# Autodesk Inventor assembly: 110033226_iam_11_農田
(part 2 of 2)
- 貼合:17 [Mate]: 110033226_ipt_44_農田基地:3 ↔ 110033226_ipt_21_柵欄:16
- 貼合:18 [Mate]: 110033226_ipt_44_農田基地:3 ↔ 110033226_ipt_21_柵欄:14
- 貼合:19 [Mate]: 110033226_ipt_44_農田基地:3 ↔ 110033226_ipt_21_柵欄:14
- 貼合:20 [Mate]: 110033226_ipt_04_小河:3 ↔ 110033226_ipt_21_柵欄:14
- 貼合:21 [Mate]: 110033226_ipt_44_農田基地:3 ↔ 110033226_ipt_21_柵欄:15
- 貼合:22 [Mate]: 110033226_ipt_44_農田基地:3 ↔ 110033226_ipt_21_柵欄:15
- 貼合:23 [Mate]: 110033226_ipt_04_小河:15 ↔ 110033226_ipt_21_柵欄:15
- 貼合:24 [Mate]: 110033226_ipt_44_農田基地:3 ↔ 110033226_ipt_07_磚塊樺木(2x1):1
- 貼合:25 [Mate]: 110033226_ipt_44_農田基地:3 ↔ 110033226_ipt_07_磚塊樺木(2x1):1
- 貼合:26 [Mate]: 110033226_ipt_44_農田基地:3 ↔ 110033226_ipt_07_磚塊樺木(2x1):1
- 貼合:27 [Mate]: 110033226_ipt_44_農田基地:3 ↔ 110033226_ipt_07_磚塊樺木(2x1):3
- 貼合:28 [Mate]: 110033226_ipt_44_農田基地:3 ↔ 110033226_ipt_07_磚塊樺木(2x1):3
- 貼合:29 [Mate]: 110033226_ipt_44_農田基地:3 ↔ 110033226_ipt_07_磚塊樺木(2x1):3
- 貼合:30 [Mate]: 110033226_ipt_44_農田基地:3 ↔ 110033226_ipt_07_磚塊樺木(2x1):5
- 貼合:31 [Mate]: 110033226_ipt_44_農田基地:3 ↔ 110033226_ipt_07_磚塊樺木(2x1):5
- 貼合:32 [Mate]: 110033226_ipt_44_農田基地:3 ↔ 110033226_ipt_07_磚塊樺木(2x1):5
- 貼合:33 [Mate]: 110033226_ipt_44_農田基地:3 ↔ 110033226_ipt_07_磚塊樺木(2x1):2
- 貼合:34 [Mate]: 110033226_ipt_44_農田基地:3 ↔ 110033226_ipt_07_磚塊樺木(2x1):2
- 貼合:35 [Mate]: 110033226_ipt_44_農田基地:3 ↔ 110033226_ipt_07_磚塊樺木(2x1):2
- 貼合:36 [Mate]: 110033226_ipt_44_農田基地:3 ↔ 110033226_ipt_07_磚塊樺木(2x1):4
- 貼合:37 [Mate]: 110033226_ipt_44_農田基地:3 ↔ 110033226_ipt_07_磚塊樺木(2x1):4
- 貼合:38 [Mate]: 110033226_ipt_44_農田基地:3 ↔ 110033226_ipt_07_磚塊樺木(2x1):4
- 貼合:39 [Mate]: 110033226_ipt_44_農田基地:3 ↔ 110033226_ipt_13_草地二:1
- 貼合:40 [Mate]: 110033226_ipt_44_農田基地:3 ↔ 110033226_ipt_13_草地二:1
- 貼合:41 [Mate]: 110033226_ipt_44_農田基地:3 ↔ 110033226_ipt_13_草地二:1
- 貼合:42 [Mate]: 110033226_ipt_44_農田基地:3 ↔ 110033226_ipt_13_草地二:12
- 貼合:43 [Mate]: 110033226_ipt_44_農田基地:3 ↔ 110033226_ipt_13_草地二:12
- 貼合:44 [Mate]: 110033226_ipt_44_農田基地:3 ↔ 110033226_ipt_13_草地二:12
- 貼合:45 [Mate]: 110033226_ipt_44_農田基地:3 ↔ 110033226_ipt_13_草地二:11
- 貼合:46 [Mate]: 110033226_ipt_44_農田基地:3 ↔ 110033226_ipt_13_草地二:11
- 貼合:47 [Mate]: 110033226_ipt_44_農田基地:3 ↔ 110033226_ipt_13_草地二:11
- 貼合:48 [Mate]: 110033226_ipt_44_農田基地:3 ↔ 110033226_ipt_07_磚塊樺木(2x1):38
- 貼合:49 [Mate]: 110033226_ipt_44_農田基地:3 ↔ 110033226_ipt_07_磚塊樺木(2x1):38
- 貼合:50 [Mate]: 110033226_ipt_44_農田基地:3 ↔ 110033226_ipt_06_磚塊樺木(1x1):3
- 貼合:51 [Mate]: 110033226_ipt_07_磚塊樺木(2x1):38 ↔ 110033226_ipt_06_磚塊樺木(1x1):3
- 貼合:52 [Mate]: 110033226_ipt_07_磚塊樺木(2x1):38 ↔ 110033226_ipt_06_磚塊樺木(1x1):3
- 貼合:53 [Mate]: 110033226_ipt_06_磚塊樺木(1x1):11 ↔ 110033226_ipt_07_磚塊樺木(2x1):36
- 貼合:54 [Mate]: 110033226_ipt_06_磚塊樺木(1x1):11 ↔ 110033226_ipt_07_磚塊樺木(2x1):36
- 貼合:55 [Mate]: 110033226_ipt_07_磚塊樺木(2x1):46 ↔ 110033226_ipt_07_磚塊樺木(2x1):36
- 貼合:56 [Mate]: 110033226_ipt_07_磚塊樺木(2x1):46 ↔ 110033226_ipt_06_磚塊樺木(1x1):1
- 貼合:57 [Mate]: 110033226_ipt_07_磚塊樺木(2x1):36 ↔ 110033226_ipt_06_磚塊樺木(1x1):1
- 貼合:58 [Mate]: 110033226_ipt_07_磚塊樺木(2x1):36 ↔ 110033226_ipt_06_磚塊樺木(1x1):1
- 貼合:59 [Mate]: 110033226_ipt_06_磚塊樺木(1x1):10 ↔ 110033226_ipt_07_磚塊樺木(2x1):37
- 貼合:60 [Mate]: 110033226_ipt_06_磚塊樺木(1x1):9 ↔ 110033226_ipt_07_磚塊樺木(2x1):37
- 貼合:61 [Mate]: 110033226_ipt_06_磚塊樺木(1x1):10 ↔ 110033226_ipt_07_磚塊樺木(2x1):37
- 貼合:62 [Mate]: 110033226_ipt_06_磚塊樺木(1x1):8 ↔ 110033226_ipt_06_磚塊樺木(1x1):2
- 貼合:63 [Mate]: 110033226_ipt_06_磚塊樺木(1x1):8 ↔ 110033226_ipt_06_磚塊樺木(1x1):2
- 貼合:64 [Mate]: 110033226_ipt_06_磚塊樺木(1x1):8 ↔ 110033226_ipt_06_磚塊樺木(1x1):2
- 貼合:65 [Mate]: 110033226_ipt_06_磚塊樺木(1x1):96 ↔ 110033226_ipt_07_磚塊樺木(2x1):144
- 貼合:66 [Mate]: 110033226_ipt_06_磚塊樺木(1x1):96 ↔ 110033226_ipt_07_磚塊樺木(2x1):144
- 貼合:67 [Mate]: 110033226_ipt_07_磚塊樺木(2x1):143 ↔ 110033226_ipt_07_磚塊樺木(2x1):144
- 貼合:68 [Mate]: 110033226_ipt_07_磚塊樺木(2x1):65 ↔ 110033226_ipt_07_磚塊樺木(2x1):184
- 貼合:69 [Mate]: 110033226_ipt_07_磚塊樺木(2x1):56 ↔ 110033226_ipt_07_磚塊樺木(2x1):184
- 貼合:70 [Mate]: 110033226_ipt_07_磚塊樺木(2x1):65 ↔ 110033226_ipt_07_磚塊樺木(2x1):184
- 貼合:71 [Mate]: 110033226_ipt_07_磚塊樺木(2x1):56 ↔ 110033226_ipt_06_磚塊樺木(1x1):133
- 貼合:72 [Mate]: 110033226_ipt_07_磚塊樺木(2x1):56 ↔ 110033226_ipt_06_磚塊樺木(1x1):133
- 貼合:73 [Mate]: 110033226_ipt_07_磚塊樺木(2x1):56 ↔ 110033226_ipt_06_磚塊樺木(1x1):133
- 貼合:74 [Mate]: 110033226_ipt_07_磚塊樺木(2x1):84 ↔ 110033226_ipt_12_平滑面(2x1):1
- 貼合:75 [Mate]: 110033226_ipt_07_磚塊樺木(2x1):84 ↔ 110033226_ipt_12_平滑面(2x1):1
- 貼合:76 [Mate]: 110033226_ipt_07_磚塊樺木(2x1):84 ↔ 110033226_ipt_12_平滑面(2x1):1
- 貼合:77 [Mate]: 110033226_ipt_07_磚塊樺木(2x1):38 ↔ 110033226_ipt_08_平滑面(3x1):1
- 貼合:78 [Mate]: 110033226_ipt_07_磚塊樺木(2x1):47 ↔ 110033226_ipt_08_平滑面(3x1):1
- 貼合:79 [Mate]: 110033226_ipt_08_平滑面(3x1):1 ↔ 110033226_ipt_06_磚塊樺木(1x1):97
- 貼合:80 [Mate]: 110033226_ipt_07_磚塊樺木(2x1):47 ↔ 110033226_ipt_08_平滑面(3x1):9
- 貼合:81 [Mate]: 110033226_ipt_07_磚塊樺木(2x1):47 ↔ 110033226_ipt_08_平滑面(3x1):9
- 貼合:82 [Mate]: 110033226_ipt_06_磚塊樺木(1x1):26 ↔ 110033226_ipt_08_平滑面(3x1):11
- 貼合:83 [Mate]: 110033226_ipt_06_磚塊樺木(1x1):50 ↔ 110033226_ipt_08_平滑面(3x1):11
- 貼合:84 [Mate]: 110033226_ipt_06_磚塊樺木(1x1):50 ↔ 110033226_ipt_08_平滑面(3x1):11
- 貼合:85 [Mate]: 110033226_ipt_07_磚塊樺木(2x1):54 ↔ 110033226_ipt_07_磚塊樺木(2x1):208
- 貼合:86 [Mate]: 110033226_ipt_07_磚塊樺木(2x1):53 ↔ 110033226_ipt_07_磚塊樺木(2x1):208
- 貼合:87 [Mate]: 110033226_ipt_07_磚塊樺木(2x1):54 ↔ 110033226_ipt_07_磚塊樺木(2x1):208
- 貼合:88 [Mate]: 110033226_ipt_44_農田基地:3 ↔ 110033226_ipt_38_小樹木:2
- 貼合:89 [Mate]: 110033226_ipt_44_農田基地:3 ↔ 110033226_ipt_38_小樹木:2
- 貼合:90 [Mate]: 110033226_ipt_44_農田基地:3 ↔ 110033226_ipt_38_小樹木:2
- 貼合:91 [Mate]: 110033226_ipt_38_小樹木:1 ↔ 110033226_ipt_44_農田基地:3
- 貼合:92 [Mate]: 110033226_ipt_38_小樹木:1 ↔ 110033226_ipt_44_農田基地:3
- 貼合:93 [Mate]: 110033226_ipt_38_小樹木:1 ↔ 110033226_ipt_44_農田基地:3
- 貼合:94 [Mate]: 110033226_ipt_44_農田基地:3 ↔ 110033226_ipt_38_小樹木:5
- 貼合:95 [Mate]: 110033226_ipt_44_農田基地:3 ↔ 110033226_ipt_38_小樹木:5
- 貼合:96 [Mate]: 110033226_ipt_38_小樹木:1 ↔ 110033226_ipt_38_小樹木:5
- 貼合:97 [Mate]: 110033226_ipt_44_農田基地:3 ↔ 110033226_ipt_38_小樹木:4
- 對稱:1 [Symmetry]: 110033226_ipt_38_小樹木:3 ↔ 110033226_ipt_38_小樹木:4
- 貼合:98 [Mate]: 110033226_ipt_44_農田基地:3 ↔ 110033226_ipt_38_小樹木:4
- 貼合:99 [Mate]: 110033226_ipt_45_小農田基地:1 ↔ 110033226_ipt_44_農田基地:1
- 貼合:100 [Mate]: 110033226_ipt_45_小農田基地:1 ↔ 110033226_ipt_44_農田基地:1
- 貼合:101 [Mate]: 110033226_ipt_45_小農田基地:1 ↔ 110033226_ipt_44_農田基地:1
- 貼合:102 [Mate]: 110033226_ipt_45_小農田基地:1 ↔ 110033226_ipt_04_小河:26
- 貼合:103 [Mate]: 110033226_ipt_45_小農田基地:1 ↔ 110033226_ipt_04_小河:26
- 貼合:104 [Mate]: 110033226_ipt_45_小農田基地:1 ↔ 110033226_ipt_04_小河:26
- 貼合:105 [Mate]: 110033226_ipt_45_小農田基地:1 ↔ 110033226_ipt_21_柵欄:49
- 貼合:106 [Mate]: 110033226_ipt_45_小農田基地:1 ↔ 110033226_ipt_21_柵欄:49
- 貼合:107 [Mate]: 110033226_ipt_45_小農田基地:1 ↔ 110033226_ipt_21_柵欄:49
- 貼合:108 [Mate]: 110033226_ipt_45_小農田基地:1 ↔ 110033226_ipt_21_柵欄:50
- 貼合:109 [Mate]: 110033226_ipt_45_小農田基地:1 ↔ 110033226_ipt_21_柵欄:50
- 貼合:110 [Mate]: 110033226_ipt_45_小農田基地:1 ↔ 110033226_ipt_21_柵欄:50
- 貼合:111 [Mate]: 110033226_ipt_45_小農田基地:1 ↔ 110033226_ipt_11_樓梯支架:1
- 貼合:112 [Mate]: 110033226_ipt_45_小農田基地:1 ↔ 110033226_ipt_11_樓梯支架:1
- 貼合:113 [Mate]: 110033226_ipt_45_小農田基地:1 ↔ 110033226_ipt_11_樓梯支架:1
- 貼合:114 [Mate]: 110033226_ipt_11_樓梯支架:12 ↔ 110033226_ipt_08_平滑面(3x1):25
- 貼合:115 [Mate]: 110033226_ipt_11_樓梯支架:12 ↔ 110033226_ipt_08_平滑面(3x1):25
- 貼合:116 [Mate]: 110033226_ipt_11_樓梯支架:12 ↔ 110033226_ipt_08_平滑面(3x1):25
- 貼合:117 [Mate]: 110033226_ipt_11_樓梯支架:8 ↔ 110033226_ipt_08_平滑面(3x1):32
- 貼合:118 [Mate]: 110033226_ipt_11_樓梯支架:9 ↔ 110033226_ipt_08_平滑面(3x1):30
- 貼合:119 [Mate]: 110033226_ipt_11_樓梯支架:5 ↔ 110033226_ipt_08_平滑面(3x1):31
- 貼合:120 [Mate]: 110033226_ipt_11_樓梯支架:6 ↔ 110033226_ipt_08_平滑面(3x1):28
- 貼合:121 [Mate]: 110033226_ipt_11_樓梯支架:12 ↔ 110033226_ipt_08_平滑面(3x1):29
- 貼合:122 [Mate]: 110033226_ipt_08_平滑面(3x1):26 ↔ 110033226_ipt_08_平滑面(3x1):27
- 貼合:123 [Mate]: 110033226_ipt_08_平滑面(3x1):26 ↔ 110033226_ipt_08_平滑面(3x1):27
- 貼合:124 [Mate]: 110033226_ipt_08_平滑面(3x1):26 ↔ 110033226_ipt_08_平滑面(3x1):27
- 貼合:125 [Mate]: 110033226_ipt_11_樓梯支架:12 ↔ 110033226_ipt_08_平滑面(3x1):29
- 貼合:126 [Mate]: 110033226_ipt_11_樓梯支架:6 ↔ 110033226_ipt_08_平滑面(3x1):28
- 貼合:127 [Mate]: 110033226_ipt_11_樓梯支架:5 ↔ 110033226_ipt_08_平滑面(3x1):31
- 貼合:128 [Mate]: 110033226_ipt_11_樓梯支架:9 ↔ 110033226_ipt_08_平滑面(3x1):30
- 貼合:129 [Mate]: 110033226_ipt_11_樓梯支架:8 ↔ 110033226_ipt_08_平滑面(3x1):32
- 貼合:130 [Mate]: 110033226_ipt_45_小農田基地:1 ↔ 110033226_ipt_04_小河:29
- 貼合:131 [Mate]: 110033226_ipt_45_小農田基地:1 ↔ 110033226_ipt_04_小河:29
- 貼合:132 [Mate]: 110033226_ipt_04_小河:47 ↔ 110033226_ipt_04_小河:56
- 貼合:133 [Mate]: 110033226_ipt_04_小河:47 ↔ 110033226_ipt_04_小河:56
- 貼合:134 [Mate]: 110033226_ipt_04_小河:47 ↔ 110033226_ipt_04_小河:56
- 貼合:135 [Mate]: 110033226_ipt_45_小農田基地:1 ↔ 110033226_ipt_04_小河:63
- 貼合:136 [Mate]: 110033226_ipt_45_小農田基地:1 ↔ 110033226_ipt_04_小河:63
- 貼合:137 [Mate]: 110033226_ipt_45_小農田基地:1 ↔ 110033226_ipt_04_小河:63
- 貼合:138 [Mate]: 110033226_ipt_45_小農田基地:1 ↔ 110033226_ipt_04_小河:64
- 貼合:139 [Mate]: 110033226_ipt_45_小農田基地:1 ↔ 110033226_ipt_04_小河:64
- 貼合:140 [Mate]: 110033226_ipt_45_小農田基地:1 ↔ 110033226_ipt_04_小河:64
- 貼合:141 [Mate]: 110033226_ipt_45_小農田基地:1 ↔ 110033226_ipt_37_小河方塊:1
- 貼合:142 [Mate]: 110033226_ipt_45_小農田基地:1 ↔ 110033226_ipt_37_小河方塊:1
- 貼合:143 [Mate]: 110033226_ipt_04_小河:67 ↔ 110033226_ipt_37_小河方塊:1
- 貼合:144 [Mate]: 110033226_ipt_04_小河:32 ↔ 110033226_ipt_37_小河方塊:5
- 貼合:145 [Mate]: 110033226_ipt_04_小河:32 ↔ 110033226_ipt_37_小河方塊:5
- 貼合:146 [Mate]: 110033226_ipt_45_小農田基地:1 ↔ 110033226_ipt_37_小河方塊:5
- 貼合:147 [Mate]: 110033226_ipt_04_小河:34 ↔ 110033226_ipt_04_小河:68
- 貼合:148 [Mate]: 110033226_ipt_45_小農田基地:1 ↔ 110033226_ipt_04_小河:68
- 貼合:149 [Mate]: 110033226_ipt_04_小河:35 ↔ 110033226_ipt_04_小河:68
- 貼合:150 [Mate]: 110033226_ipt_02_草地一:1 ↔ 110033226_ipt_04_小河:82
- 貼合:151 [Mate]: 110033226_ipt_02_草地一:1 ↔ 110033226_ipt_04_小河:82
- 貼合:153 [Mate]: 110033226_ipt_02_草地一:3 ↔ 110033226_ipt_04_小河:73
- 貼合:154 [Mate]: 110033226_ipt_02_草地一:2 ↔ 110033226_ipt_38_小樹木:24
- 貼合:155 [Mate]: 110033226_ipt_02_草地一:2 ↔ 110033226_ipt_38_小樹木:24
- 貼合:156 [Mate]: 110033226_ipt_02_草地一:2 ↔ 110033226_ipt_38_小樹木:24
- 貼合:157 [Mate]: 110033226_ipt_02_草地一:2 ↔ 110033226_ipt_38_小樹木:23
- 貼合:158 [Mate]: 110033226_ipt_02_草地一:2 ↔ 110033226_ipt_38_小樹木:23
- 貼合:159 [Mate]: 110033226_ipt_02_草地一:2 ↔ 110033226_ipt_38_小樹木:23
